# Autodesk Inventor assembly: mini_3pi_caster_wheel
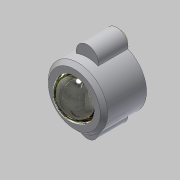
[picture p0: Inventor's stored thumbnail of the model, 180x180]
Saved by Autodesk Inventor 2019.3 (Build 233278000, 278)
## iProperties
Created: 2019-03-11
Part Number: mini_3pi_caster_wheel
Document SubType Name: Assembly
Designer: Varga Daniel
Author: Varga Daniel
## Documents named in this file (4)
- C:\!_Dani\!_cloud\OneDrive\!_munka\Revolution\RevvyDemoKit\Structural parts\Demo parts\Caster wheel\Inventor imported\mini_3pi_caster_wheel.iam
- C:\!_Dani\!_cloud\OneDrive\!_munka\Revolution\RevvyDemoKit\Structural parts\Demo parts\Caster wheel\Inventor imported\mini_3pi_caster_ball.ipt
- C:\!_Dani\!_cloud\OneDrive\!_munka\Revolution\RevvyDemoKit\Structural parts\Demo parts\Caster wheel\Inventor imported\mini_3pi_caster_body.ipt
- C:\!_Dani\!_cloud\OneDrive\!_dokumentumok\Inventor\Content Center Files\R2019\en-US\ISO 7049 - C-Z(2)\ISO 7049 - ST 2,2 x 6,5 - C - Z.ipt
## Components (4 placed, 3 different names)
1. mini_3pi_caster_ball:1 — Mate:3, Tangent:1
2. mini_3pi_caster_body:1 — Mate:1, Flush:1, Mate:2, Mate:3, Angle:1, Flush:5, Insert:1, Insert:2
3. ISO 7049 - C-Z ST 2,2 x 6,5 - C - Z:1 — Insert:2
4. ISO 7049 - C-Z ST 2,2 x 6,5 - C - Z:2 — Insert:1
## Relationships (9: Mate 3, Flush 2, Insert 2, Angle 1, Tangent 1)
- Mate:1: mini_3pi_caster_body:1
- Flush:1: mini_3pi_caster_body:1
- Mate:2: mini_3pi_caster_body:1
- Mate:3: mini_3pi_caster_ball:1 ↔ mini_3pi_caster_body:1
- Angle:1 (0 deg): mini_3pi_caster_body:1
- Tangent:1: mini_3pi_caster_ball:1
- Flush:5 (14.8 mm): mini_3pi_caster_body:1
- Insert:1: mini_3pi_caster_body:1 ↔ ISO 7049 - C-Z ST 2,2 x 6,5 - C - Z:2
- Insert:2: mini_3pi_caster_body:1 ↔ ISO 7049 - C-Z ST 2,2 x 6,5 - C - Z:1
